# Autodesk Inventor assembly: Peg toy assembly
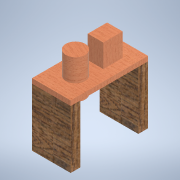
[picture p0: Inventor's stored thumbnail of the model, 180x180]
Saved by Autodesk Inventor 2021 (Build 250183000, 183)
## iProperties
Created: 2020-05-07
Part Number: Peg toy assembly
Document SubType Name: Assembly
Designer: david
Author: david
## Documents named in this file (5)
- C:\Users\david\Documents\Inventor\Peg toy assembly.iam
- C:\Users\david\Documents\Inventor\peg toy (top board)[holy].ipt
- C:\Users\david\Documents\Inventor\circle peg.ipt
- C:\Users\david\Documents\Inventor\square peg.ipt
- C:\Users\david\Documents\Inventor\peg toy (leg).ipt
## Components (5 placed, 4 different names)
1. peg toy (top board)[holy]:1 — Mate:2, Mate:3, Mate:4, Flush:1, Flush:2, Mate:5, Flush:3, Flush:4, Mate:6
2. circle peg:1 — Mate:6
3. square peg:1 — Mate:2, Mate:3
4. peg toy (leg):1 — Mate:4, Flush:1, Flush:2
5. peg toy (leg):2 — Mate:5, Flush:3, Flush:4
## Relationships (9: Mate 5, Flush 4)
- Mate:2: peg toy (top board)[holy]:1 ↔ square peg:1
- Mate:3: peg toy (top board)[holy]:1 ↔ square peg:1
- Mate:4: peg toy (top board)[holy]:1 ↔ peg toy (leg):1
- Flush:1: peg toy (top board)[holy]:1 ↔ peg toy (leg):1
- Flush:2: peg toy (top board)[holy]:1 ↔ peg toy (leg):1
- Mate:5: peg toy (top board)[holy]:1 ↔ peg toy (leg):2
- Flush:3: peg toy (top board)[holy]:1 ↔ peg toy (leg):2
- Flush:4: peg toy (top board)[holy]:1 ↔ peg toy (leg):2
- Mate:6: peg toy (top board)[holy]:1 ↔ circle peg:1
